# Autodesk Inventor assembly: Flexiwheel with Hub
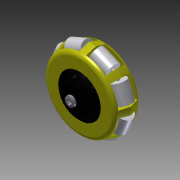
[picture p0: Inventor's stored thumbnail of the model, 180x180]
Saved by Autodesk Inventor 2014 (Build 180170000, 170)
## iProperties
Created: 2014-02-14
Part Number: Flexiwheel with Hub
Document SubType Name: Assembly
Designer: Spooner
Author: Spooner
## Documents named in this file (5)
- C:\Users\Spooner\Documents\Inventor\FerretBall Robot\3Pod\Inventor 2014 Files\Flexiwheel with Hub.iam
- C:\Users\Spooner\Documents\Inventor\FerretBall Robot\3Pod\Inventor 2014 Files\Flexiwheel Hub - Motor Side.ipt
- C:\Users\Spooner\Documents\Inventor\FerretBall Robot\3Pod\Inventor 2014 Files\Flexiwheel Hub - Out Side.ipt
- C:\Users\Spooner\Documents\Inventor\FerretBall Robot\3Pod\Inventor 2014 Files\Flexiwheel.iam
- C:\Users\Spooner\Documents\Inventor\Content Center Files\R2014\en-US\JIS B 1111(1)\JIS B 1111 - M3x6(1).ipt
## Components (4 placed, 4 different names)
1. Flexiwheel Hub - Motor Side:1 — Insert:2, Mate:2
2. Flexiwheel Hub - Out Side:1 — Insert:1, Mate:1, Insert:3
3. Flexiwheel:1 [sub-assembly] — Insert:1, Mate:1, Insert:2, Mate:2
4. JIS B 1111 M3x6:1 — Insert:3
## Relationships (5: Insert 3, Mate 2)
- Insert:1: Flexiwheel Hub - Out Side:1 ↔ Flexiwheel:1
- Mate:1: Flexiwheel Hub - Out Side:1 ↔ Flexiwheel:1
- Insert:2: Flexiwheel Hub - Motor Side:1 ↔ Flexiwheel:1
- Mate:2: Flexiwheel Hub - Motor Side:1 ↔ Flexiwheel:1
- Insert:3: Flexiwheel Hub - Out Side:1 ↔ JIS B 1111 M3x6:1
